# Autodesk Inventor assembly: MG_996R
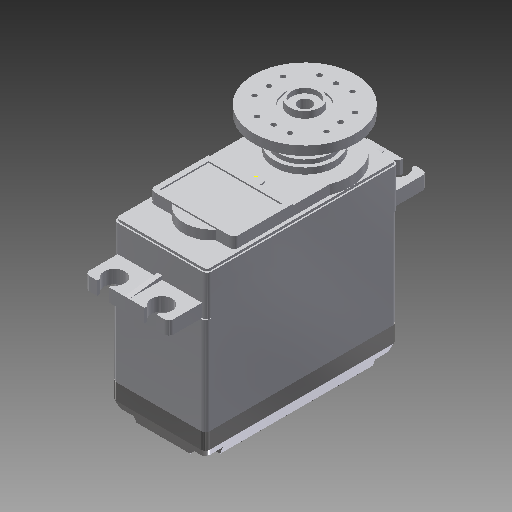
[picture p0: Inventor's stored thumbnail of the model, 512x512]
Saved by Autodesk Inventor 2018 (Build 220112000, 112)
## iProperties
Created: 2016-09-26
Part Number: MG_996R
Document SubType Name: Assembly
Designer: Julian
Mass: 55 g
Surface Area: 116.519 cm^2
Volume: 31.2727 cm^3
Author: Julian
## Documents named in this file (6)
- D:\Users\Thomas\Desktop\Projet robot augmenté\armConcept_v1\MG996R SERVO\MG_996R.iam
- D:\Users\Thomas\Desktop\Projet robot augmenté\armConcept_v1\MG996R SERVO\Base.ipt
- D:\Users\Thomas\Desktop\Projet robot augmenté\armConcept_v1\MG996R SERVO\Medio.ipt
- D:\Users\Thomas\Desktop\Projet robot augmenté\armConcept_v1\MG996R SERVO\Top.ipt
- D:\Users\Thomas\Desktop\Projet robot augmenté\armConcept_v1\MG996R SERVO\Eje.ipt
- D:\Users\Thomas\Desktop\Projet robot augmenté\armConcept_v1\MG996R SERVO\Acople circular.ipt
## Components (5 placed, 5 different names)
1. Top:1 — Rígido:2, De rotación:1
2. Medio:1 — Rígido:1, Rígido:2
3. Base:1 — Rígido:1
4. Eje:1 — De rotación:1, De rotación:2
5. Acople circular:1 — De rotación:2
## Relationships (4: WeldJoint 2, RevoluteJoint 2)
- Rígido:1 [WeldJoint]: Medio:1 ↔ Base:1
- Rígido:2 [WeldJoint]: Top:1 ↔ Medio:1
- De rotación:1 [RevoluteJoint]: Top:1 ↔ Eje:1
- De rotación:2 [RevoluteJoint]: Eje:1 ↔ Acople circular:1
